# Autodesk Inventor assembly: Alliance Short Mogo
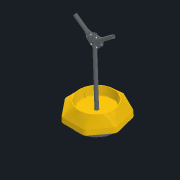
[picture p0: Inventor's stored thumbnail of the model, 180x180]
Saved by Autodesk Inventor 2021 (Build 250183000, 183)
## iProperties
Created: 2021-05-29
Part Number: Alliance Short Mogo
Document SubType Name: Assembly
Designer: max
Sending System: Autodesk Inventor 2021
Preprocessor: ST-DEVELOPER v18.1
Title: C:\Users\max\Desktop\Vex\TiP FieldCAD\Mogos\Alliance Short Mogo.stp
Author: max
Revision Number: ANY
## Documents named in this file (11)
- C:\Users\max\Desktop\Vex\TiP FieldCAD\Mogos\Neutral Short Mogo.iam
- C:\Users\max\Desktop\Vex\TiP FieldCAD\Mogos\Screw 8-32 Steel .375.ipt
- C:\Users\max\Desktop\Vex\TiP FieldCAD\Mogos\Nut Nylock.ipt
- C:\Users\max\Desktop\Vex\TiP FieldCAD\Mogos\Mogo Branch Splitter.ipt
- C:\Users\max\Desktop\Vex\TiP FieldCAD\Mogos\Mogo Branch.ipt
- C:\Users\max\Desktop\Vex\TiP FieldCAD\Mogos\Mogo Post.ipt
- C:\Users\max\Desktop\Vex\TiP FieldCAD\Mogos\Mogo Base Post Grip.ipt
- C:\Users\max\Desktop\Vex\TiP FieldCAD\Mogos\Mogo Base Yellow.ipt
- C:\Users\max\Desktop\Vex\TiP FieldCAD\Mogos\Screw 8-32 Steel .625.ipt
- C:\Users\max\Desktop\Vex\TiP FieldCAD\Mogos\Mogo Base Bottom.ipt
- C:\Users\max\Desktop\Vex\TiP FieldCAD\Mogos\Mogo Base Weight.ipt
## Components (29 placed, 10 different names)
1. Screw 8-32 Steel .375:1
2. Nut Nylock:1
3. Mogo Branch Splitter:1
4. Mogo Branch:1
5. Mogo Post:1 — Mate:2
6. Mogo Branch:2
7. Mogo Branch Splitter:2
8. Screw 8-32 Steel .375:2
9. Nut Nylock:2
10. Screw 8-32 Steel .375:3
11. Nut Nylock:3
12. Screw 8-32 Steel .375:4
13. Nut Nylock:4
14. Screw 8-32 Steel .375:5
15. Nut Nylock:5
16. Screw 8-32 Steel .375:6
17. Nut Nylock:6
18. Mogo Base Post Grip:1
19. Mogo Base Yellow:1
20. Mogo Base Post Grip:2
21. Nut Nylock:7
22. Screw 8-32 Steel .625:7
23. Nut Nylock:8
24. Screw 8-32 Steel .625:8
25. Nut Nylock:9
26. Nut Nylock:10
27. Nut Nylock:11
28. Mogo Base Bottom:1 — Mate:1, Mate:3
29. Mogo Base Weight:1 — Mate:1, Mate:2, Mate:3
## Relationships (3: Mate 3)
- Mate:1: Mogo Base Bottom:1 ↔ Mogo Base Weight:1
- Mate:2: Mogo Post:1 ↔ Mogo Base Weight:1
- Mate:3: Mogo Base Bottom:1 ↔ Mogo Base Weight:1
